# Autodesk Inventor assembly: Box_Assembly
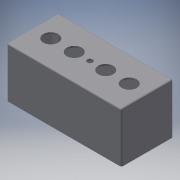
[picture p0: Inventor's stored thumbnail of the model, 180x180]
Saved by Autodesk Inventor 2018.3 (Build 223285000, 285)
## iProperties
Created: 2022-01-12
Part Number: Box_Assembly
Document SubType Name: Assembly
Designer: Michael
Author: Michael
## Documents named in this file (3)
- C:\Users\Michael\Documents\Github\nixie_clock\Inventor\Box_Assembly.iam
- C:\Users\Michael\Documents\Github\nixie_clock\Inventor\Box.ipt
- C:\Users\Michael\Documents\Github\nixie_clock\Inventor\Cover.ipt
## Components (2 placed, 2 different names)
1. Box:1 — Mate:1, Mate:2, Mate:3
2. Cover:1 — Mate:1, Mate:2, Mate:3
## Relationships (3: Mate 3)
- Mate:1: Box:1 ↔ Cover:1
- Mate:2: Box:1 ↔ Cover:1
- Mate:3: Box:1 ↔ Cover:1
